# Autodesk Inventor assembly: LIA0006-ARDUINO SHELF
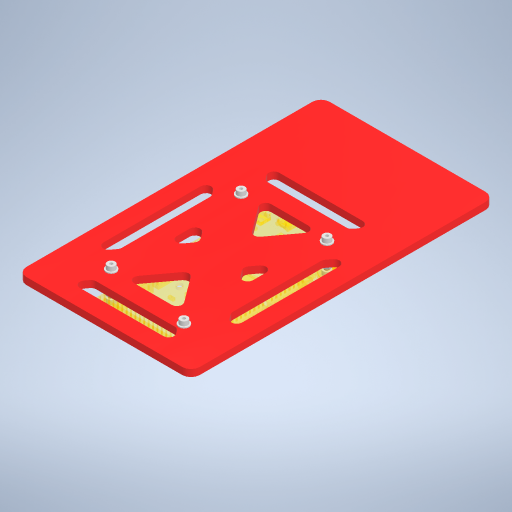
[picture p0: Inventor's stored thumbnail of the model, 512x512]
Saved by Autodesk Inventor 2023 (Build 270158000, 158)
## iProperties
Created: 2023-05-05
Part Number: LIA0006-ARDUINO SHELF
Document SubType Name: Assembly
Designer: Louis
Author: Louis
## Documents named in this file (6)
- D:\Louis\Documents\Inventor\Interferometry\LIA0006-ARDUINO SHELF.iam
- D:\Louis\Documents\Inventor\Interferometry\LI0014-ARDUINO SHELF.ipt
- D:\Louis\Documents\Inventor\Interferometry\M2.5 WASHER.ipt
- D:\Louis\Documents\Inventor\Interferometry\M2.5 X 6.ipt
- D:\Louis\Documents\Inventor\Interferometry\ACCU HHTPS-M2.5-5-8-S-Z.ipt
- D:\Louis\Documents\Inventor\Interferometry\ARDUINO DUE_Simplify.ipt
## Components (18 placed, 5 different names)
1. LI0014-ARDUINO SHELF:1 — Mate:1, Mate:2, Mate:3, Insert:1, Insert:2, Insert:3, Insert:4, Insert:9, Insert:10, Insert:11, Insert:12, Angle:1
2. M2.5 WASHER:1 — Insert:1, Insert:5
3. M2.5 WASHER:2 — Insert:4, Insert:8
4. M2.5 WASHER:3 — Insert:2, Insert:6
5. M2.5 WASHER:4 — Insert:3, Insert:7
6. M2.5 X 6:1 — Insert:6
7. M2.5 X 6:2
8. M2.5 X 6:3 — Insert:5
9. M2.5 X 6:4 — Insert:8
10. M2.5 X 6:5 — Insert:7
11. M2.5 X 6:6
12. M2.5 X 6:7
13. M2.5 X 6:8
14. ACCU HHTPS-M2.5-5-8-S-Z:1 — Insert:12
15. ACCU HHTPS-M2.5-5-8-S-Z:2 — Insert:11, Insert:13
16. ACCU HHTPS-M2.5-5-8-S-Z:3 — Insert:10
17. ACCU HHTPS-M2.5-5-8-S-Z:4 — Insert:9
18. ARDUINO DUE_Simplify:1 — Insert:13, Angle:1
## Relationships (17: Insert 13, Mate 3, Angle 1)
- Mate:1: LI0014-ARDUINO SHELF:1
- Mate:2: LI0014-ARDUINO SHELF:1
- Mate:3: LI0014-ARDUINO SHELF:1
- Insert:1: LI0014-ARDUINO SHELF:1 ↔ M2.5 WASHER:1
- Insert:2: LI0014-ARDUINO SHELF:1 ↔ M2.5 WASHER:3
- Insert:3: LI0014-ARDUINO SHELF:1 ↔ M2.5 WASHER:4
- Insert:4: LI0014-ARDUINO SHELF:1 ↔ M2.5 WASHER:2
- Insert:5: M2.5 WASHER:1 ↔ M2.5 X 6:3
- Insert:6: M2.5 WASHER:3 ↔ M2.5 X 6:1
- Insert:7: M2.5 WASHER:4 ↔ M2.5 X 6:5
- Insert:8: M2.5 WASHER:2 ↔ M2.5 X 6:4
- Insert:9: LI0014-ARDUINO SHELF:1 ↔ ACCU HHTPS-M2.5-5-8-S-Z:4
- Insert:10: LI0014-ARDUINO SHELF:1 ↔ ACCU HHTPS-M2.5-5-8-S-Z:3
- Insert:11: LI0014-ARDUINO SHELF:1 ↔ ACCU HHTPS-M2.5-5-8-S-Z:2
- Insert:12: LI0014-ARDUINO SHELF:1 ↔ ACCU HHTPS-M2.5-5-8-S-Z:1
- Insert:13: ACCU HHTPS-M2.5-5-8-S-Z:2 ↔ ARDUINO DUE_Simplify:1
- Angle:1 (180 deg): LI0014-ARDUINO SHELF:1 ↔ ARDUINO DUE_Simplify:1
